# Autodesk Inventor assembly: 컨버터 하우징
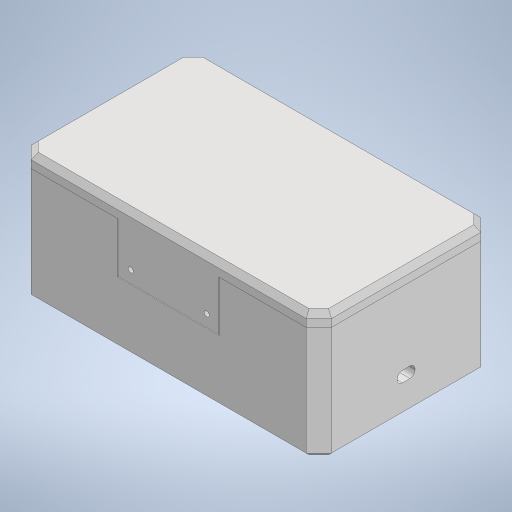
[picture p0: Inventor's stored thumbnail of the model, 512x512]
Saved by Autodesk Inventor 2023 (Build 270158000, 158)
## iProperties
Created: 2022-08-19
Part Number: 컨버터 하우징
Document SubType Name: Assembly
Designer: user
Author: user
## Documents named in this file (4)
- C:\Users\user\Desktop\PAI\PAI설계\전원 컨버터\컨버터 하우징.iam
- C:\Users\user\Desktop\PAI\PAI설계\범용 부품\AC-DC컨버터.ipt
- C:\Users\user\Desktop\PAI\PAI설계\전원 컨버터\컨버터 하우징.ipt
- C:\Users\user\Desktop\PAI\PAI설계\전원 컨버터\컨버터 커버.ipt
## Components (3 placed, 3 different names)
1. AC-DC컨버터:1 — 삽입:1, 삽입:2
2. 컨버터 하우징:1 — 삽입:1, 삽입:2, 메이트:1, 플러쉬:1
3. 컨버터 커버:1 — 메이트:1, 플러쉬:1
## Relationships (4: Insert 2, Mate 1, Flush 1)
- 삽입:1 [Insert]: AC-DC컨버터:1 ↔ 컨버터 하우징:1
- 삽입:2 [Insert]: AC-DC컨버터:1 ↔ 컨버터 하우징:1
- 메이트:1 [Mate]: 컨버터 하우징:1 ↔ 컨버터 커버:1
- 플러쉬:1 [Flush]: 컨버터 하우징:1 ↔ 컨버터 커버:1
